# Autodesk Inventor assembly: Suspension Assembly
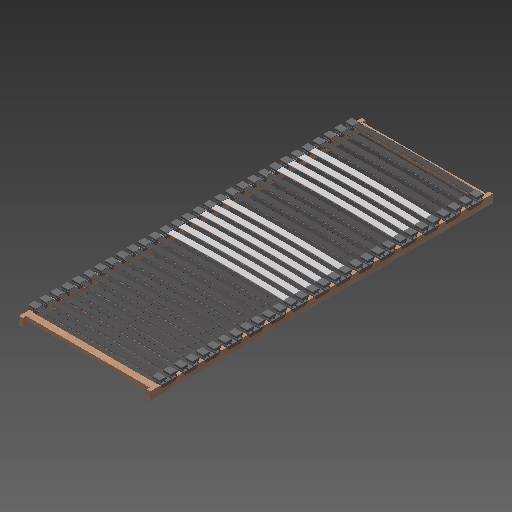
[picture p0: Inventor's stored thumbnail of the model, 512x512]
Saved by Autodesk Inventor 2017 (Build 210142000, 142)
## iProperties
Created: 2017-09-04
Part Number: Suspension Assembly
Document SubType Name: Weldment
Designer: Michael
Weld Material: Welded Aluminum-6061
Author: Michael
## Documents named in this file (6)
- C:\Users\Michael\Google Drive\Businesses\Xatie Corp\Porfolio Pieces\Hemnes Queen Bed\Suspension Assembly.iam
- C:\Users\Michael\Google Drive\Businesses\Xatie Corp\Porfolio Pieces\Hemnes Queen Bed\Rubber Damper.ipt
- C:\Users\Michael\Google Drive\Businesses\Xatie Corp\Porfolio Pieces\Hemnes Queen Bed\Suspension Board Grey.ipt
- C:\Users\Michael\Google Drive\Businesses\Xatie Corp\Porfolio Pieces\Hemnes Queen Bed\Suspension Board White.ipt
- C:\Users\Michael\Google Drive\Businesses\Xatie Corp\Porfolio Pieces\Hemnes Queen Bed\Suspension Brace.ipt
- C:\Users\Michael\Google Drive\Businesses\Xatie Corp\Porfolio Pieces\Hemnes Queen Bed\Suspension Rail.ipt
## Components (64 placed, 5 different names)
1. Suspension Brace:1 — Mate:2, Flush:1, Flush:4, Flush:5
2. Suspension Rail:1 — Mate:1, Mate:2, Flush:2, Flush:3, Flush:4, Flush:5, Flush:6, Mate:9
3. Suspension Brace:3 — Mate:1, Flush:1, Mate:3, Mate:5, Flush:6
4. Suspension Rail:2 — Mate:3, Flush:2, Flush:3, Mate:4, Mate:7, Mate:8, Mate:6
5. Suspension Board Grey:2 — Mate:10, Flush:12, Flush:14
6. Suspension Board Grey:3
7. Suspension Board Grey:4
8. Suspension Board Grey:5
9. Suspension Board Grey:6
10. Suspension Board Grey:7
11. Suspension Board Grey:8
12. Suspension Board Grey:9
13. Suspension Board Grey:10
14. Suspension Board Grey:11
15. Suspension Board Grey:12
16. Suspension Board Grey:13
17. Suspension Board Grey:1 — Mate:11, Flush:13, Flush:14, Flush:17, Flush:18
18. Suspension Board Grey:14
19. Suspension Board Grey:15
20. Suspension Board Grey:16
21. Suspension Board White:2 — Flush:15, Flush:16, Flush:17, Mate:13, Flush:19, Flush:20
22. Suspension Board White:3
23. Suspension Board White:4
24. Suspension Board White:5
25. Suspension Board White:1 — Flush:15, Flush:18, Mate:12
26. Suspension Board White:6
27. Suspension Board White:7
28. Suspension Board White:8
29. Suspension Board White:9
30. Suspension Board White:10
31. Suspension Board Grey:17 — Flush:16, Mate:14, Flush:19
32. Suspension Board Grey:18
33. Suspension Board Grey:19
34. Suspension Board Grey:20
35. Rubber Damper:1 — Mate:6, Mate:7, Mate:8
36. Rubber Damper:2
37. Rubber Damper:3
38. Rubber Damper:4
39. Rubber Damper:5
40. Rubber Damper:6
41. Rubber Damper:7
42. Rubber Damper:8
43. Rubber Damper:9
44. Rubber Damper:10
45. Rubber Damper:11
46. Rubber Damper:12
47. Rubber Damper:13
48. Rubber Damper:14
49. Rubber Damper:15
50. Rubber Damper:16
51. Rubber Damper:17 — Mate:14
52. Rubber Damper:18
53. Rubber Damper:19 — Mate:13
54. Rubber Damper:20
55. Rubber Damper:21 — Mate:11
56. Rubber Damper:22
57. Rubber Damper:23
58. Rubber Damper:24 — Mate:12
59. Rubber Damper:25
60. Rubber Damper:26
61. Rubber Damper:27
62. Rubber Damper:28
63. Rubber Damper:29
64. Rubber Damper:30 — Mate:10
## Component patterns: (2 elements), (12 elements, first: Suspension Board Grey:2), (4 elements, first: Suspension Board Grey:1), (4 elements, first: Suspension Board White:2), (6 elements, first: Suspension Board White:1), (4 elements, first: Suspension Board Grey:17), (15 elements, first: Rubber Damper:1), Component Pattern 1:2 (15 elements)
## Relationships (29: Flush 15, Mate 14)
- Mate:1: Suspension Rail:1 ↔ Suspension Brace:3
- Mate:2: Suspension Brace:1 ↔ Suspension Rail:1
- Flush:1: Suspension Brace:1 ↔ Suspension Brace:3
- Mate:3: Suspension Brace:3 ↔ Suspension Rail:2
- Flush:2: Suspension Rail:1 ↔ Suspension Rail:2
- Flush:3: Suspension Rail:1 ↔ Suspension Rail:2
- Mate:4: Suspension Rail:2
- Mate:5: Suspension Brace:3
- Flush:4: Suspension Brace:1 ↔ Suspension Rail:1
- Flush:5 (19.05 mm): Suspension Brace:1 ↔ Suspension Rail:1
- Flush:6 (-19.05 mm): Suspension Rail:1 ↔ Suspension Brace:3
- Mate:6 (-58.7375 mm): Suspension Rail:2 ↔ Rubber Damper:1
- Mate:7: Suspension Rail:2 ↔ Rubber Damper:1
- Mate:8: Suspension Rail:2 ↔ Rubber Damper:1
- Mate:9: Suspension Rail:1
- Mate:10: Suspension Board Grey:2 ↔ Rubber Damper:30
- Flush:12: Suspension Board Grey:2
- Mate:11: Suspension Board Grey:1 ↔ Rubber Damper:21
- Flush:13: Suspension Board Grey:1
- Flush:14: Suspension Board Grey:2 ↔ Suspension Board Grey:1
- Flush:15: Suspension Board White:2 ↔ Suspension Board White:1
- Flush:16: Suspension Board White:2 ↔ Suspension Board Grey:17
- Flush:17: Suspension Board Grey:1 ↔ Suspension Board White:2
- Flush:18: Suspension Board Grey:1 ↔ Suspension Board White:1
- Mate:12: Suspension Board White:1 ↔ Rubber Damper:24
- Mate:13: Suspension Board White:2 ↔ Rubber Damper:19
- Mate:14: Suspension Board Grey:17 ↔ Rubber Damper:17
- Flush:19: Suspension Board White:2 ↔ Suspension Board Grey:17
- Flush:20: Suspension Board White:2
